# Autodesk Inventor assembly: 2018RobotRhinoTrackWithRevLift
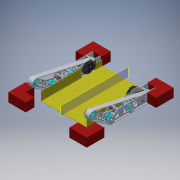
[picture p0: Inventor's stored thumbnail of the model, 180x180]
Saved by Autodesk Inventor 2019 (Build 230136000, 136)
## iProperties
Created: 2017-01-12
Part Number: 2018RobotRhinoTrackWithRevLift
Document SubType Name: Assembly
Designer: steele
Mass: 784427 g
Surface Area: 99187.8 cm^2
Volume: 668402 cm^3
Density: 1.17359 g/cm^3
Author: steele
## Documents named in this file (8)
- D:\snobotics\CAD-Development\robSteele\2018PostSeasonLift\2018RobotRhinoTrackWithRevLift.iam
- D:\snobotics\CAD-Development\robSteele\SnoBotics2017\LeftRhinoTrackAM-3322\am-3322_Rhino_Track_Drive_Module_Left.iam
- D:\snobotics\CAD-Development\robSteele\SnoBotics2017\RightRhinoTrackAM-3322\am-3322_Rhino_Track_Drive_Module_Right.iam
- D:\snobotics\CAD-Development\robSteele\SnoBotics2017\robotVolume.ipt
- D:\snobotics\CAD-Development\robSteele\SnoBotics2017\RedBumper.ipt
- D:\snobotics\CAD-Development\robSteele\SnoBotics2017\Gear\am-3302.iam
- D:\snobotics\CAD-Development\robSteele\2017CompetitionRobot\Design Accelerator\Bolted Connection1.iam
- D:\snobotics\CAD-Development\robSteele\2018PostSeasonLift\SheetBottomFloor.ipt
## Components (10 placed, 7 different names)
1. am-3322_Rhino_Track_Drive_Module_Left:1 [sub-assembly] — Mate:1, Flush:1, Flush:2, Flush:3, Flush:4, Flush:5, Mate:3, Flush:20, Flush:21, Mate:5
2. am-3322_Rhino_Track_Drive_Module_Right:1 [sub-assembly] — Mate:1, Flush:1, Flush:2, Mate:4, Mate:6, Mate:7
3. robotVolume:1 — Flush:3, Flush:4, Flush:5, Flush:14, Flush:15, Flush:18, Flush:19
4. RedBumper:1 — Mate:3
5. RedBumper:2 — Mate:4
6. RedBumper:3 — Flush:14, Flush:15
7. RedBumper:4 — Flush:18, Flush:19
8. am-3302:1 [sub-assembly]
9. SheetBottomFloor:1 — Flush:20, Flush:21, Mate:5
10. Bolted Connection:1 [sub-assembly] — Mate:6, Mate:7
## Relationships (17: Flush 11, Mate 6)
- Mate:1 (546.1 mm): am-3322_Rhino_Track_Drive_Module_Left:1 ↔ am-3322_Rhino_Track_Drive_Module_Right:1
- Flush:1: am-3322_Rhino_Track_Drive_Module_Left:1 ↔ am-3322_Rhino_Track_Drive_Module_Right:1
- Flush:2: am-3322_Rhino_Track_Drive_Module_Left:1 ↔ am-3322_Rhino_Track_Drive_Module_Right:1
- Flush:3: am-3322_Rhino_Track_Drive_Module_Left:1 ↔ robotVolume:1
- Flush:4 (106.3752 mm): am-3322_Rhino_Track_Drive_Module_Left:1 ↔ robotVolume:1
- Flush:5 (101.6 mm): am-3322_Rhino_Track_Drive_Module_Left:1 ↔ robotVolume:1
- Mate:3: am-3322_Rhino_Track_Drive_Module_Left:1 ↔ RedBumper:1
- Mate:4: am-3322_Rhino_Track_Drive_Module_Right:1 ↔ RedBumper:2
- Flush:14: robotVolume:1 ↔ RedBumper:3
- Flush:15: robotVolume:1 ↔ RedBumper:3
- Flush:18: robotVolume:1 ↔ RedBumper:4
- Flush:19: robotVolume:1 ↔ RedBumper:4
- Flush:20: am-3322_Rhino_Track_Drive_Module_Left:1 ↔ SheetBottomFloor:1
- Flush:21: am-3322_Rhino_Track_Drive_Module_Left:1 ↔ SheetBottomFloor:1
- Mate:5: am-3322_Rhino_Track_Drive_Module_Left:1 ↔ SheetBottomFloor:1
- Mate:6: am-3322_Rhino_Track_Drive_Module_Right:1 ↔ Bolted Connection:1
- Mate:7: am-3322_Rhino_Track_Drive_Module_Right:1 ↔ Bolted Connection:1
